# Autodesk Inventor assembly: Assembly1
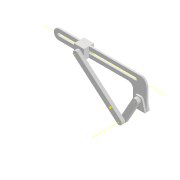
[picture p0: Inventor's stored thumbnail of the model, 180x180]
Saved by Autodesk Inventor 2021 (Build 250183000, 183)
## iProperties
Created: 2021-07-14
Part Number: Assembly1
Document SubType Name: Assembly
Designer: Santiago
Author: Santiago
## Documents named in this file (5)
- C:\Users\user\Desktop\Ingeniería Mecánica UN\6. Sexto Semestre\Métodos Numéricos\ProyectoMetodos\Simulación Inventor\Assembly1.iam
- C:\Users\user\Desktop\Ingeniería Mecánica UN\6. Sexto Semestre\Métodos Numéricos\ProyectoMetodos\Simulación Inventor\Acoplador.ipt
- C:\Users\user\Desktop\Ingeniería Mecánica UN\6. Sexto Semestre\Métodos Numéricos\ProyectoMetodos\Simulación Inventor\Bancada.ipt
- C:\Users\user\Desktop\Ingeniería Mecánica UN\6. Sexto Semestre\Métodos Numéricos\ProyectoMetodos\Simulación Inventor\Corredera.ipt
- C:\Users\user\Desktop\Ingeniería Mecánica UN\6. Sexto Semestre\Métodos Numéricos\ProyectoMetodos\Simulación Inventor\Manivela.ipt
## Components (4 placed, 4 different names)
1. Acoplador:1
2. Bancada:1
3. Corredera:1 — Mate:1, Angle:1
4. Manivela:1 — Mate:3
## Relationships (4: Mate 3, Angle 1)
- Mate:1: Corredera:1
- Angle:1 (0 deg): Corredera:1
- Mate:2
- Mate:3: Manivela:1
